# Autodesk Inventor assembly: Motor V5
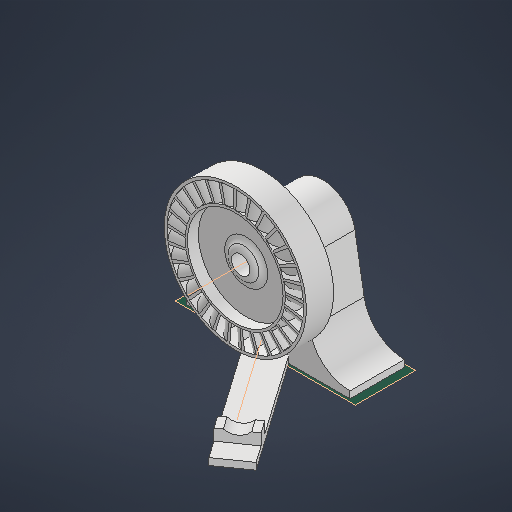
[picture p0: Inventor's stored thumbnail of the model, 512x512]
Saved by Autodesk Inventor 2025.3 (Build 293356030, 356C)
## iProperties
Created: 2025-09-23
Part Number: Motor V5
Document SubType Name: Assembly
Designer: yo
Author: yo
## Documents named in this file (3)
- C:\Users\yo\Documents\Andes\9no Semestre\Proyecto Intermedio\Proyecto\Huron-Hudson\Versions\V5\Motor V5.iam
- C:\Users\yo\Documents\Andes\9no Semestre\Proyecto Intermedio\Proyecto\Huron-Hudson\Versions\V5\Support 1 - V2.ipt
- C:\Users\yo\Documents\Andes\9no Semestre\Proyecto Intermedio\Proyecto\Huron-Hudson\Versions\V2\Pelton - V2.ipt
## Components (2 placed, 2 different names)
1. Support 1 - V2:1 — Flush:4, Flush:3, Flush:5, Mate:1, Mate:2, Mate:4
2. Pelton - V2:1 — Mate:3, Mate:4
## Relationships (7: Mate 4, Flush 3)
- Flush:4: Support 1 - V2:1
- Flush:3: Support 1 - V2:1
- Flush:5: Support 1 - V2:1
- Mate:1: Support 1 - V2:1
- Mate:2: Support 1 - V2:1
- Mate:3: Pelton - V2:1
- Mate:4 (2 mm): Support 1 - V2:1 ↔ Pelton - V2:1
